# Autodesk Inventor assembly: Front support bearing and stopper
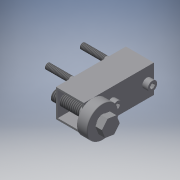
[picture p0: Inventor's stored thumbnail of the model, 180x180]
Saved by Autodesk Inventor 2018 (Build 220112000, 112)
## iProperties
Created: 2019-03-22
Part Number: Front support bearing and stopper
Document SubType Name: Assembly
Designer: s-4008082
Author: s-4008082
## Documents named in this file (6)
- \\studenthome\students\S-4008082\robotics\Front support bearing and stopper.iam
- \\studenthome\students\S-4008082\robotics\Front support bearing and stopper.ipt
- \\studenthome\students\S-4008082\robotics\10 l 20 2 1 l 2 bolt.ipt
- \\studenthome\students\S-4008082\robotics\1614zz bearing.ipt
- \\studenthome\students\S-4008082\robotics\3 l 8 Bolt.ipt
- \\studenthome\students\S-4008082\robotics\.05 spacer.ipt
## Components (7 placed, 5 different names)
1. Front support bearing and stopper:1 — Mate:4, Mate:5, Mate:6, Mate:7, Mate:9
2. 10 l 20 2 1 l 2 bolt:1 — Mate:4, Mate:7
3. 1614zz bearing:1 — Mate:8, Mate:12, Mate:14
4. 3 l 8 Bolt:1 — Mate:8, Mate:10, Mate:11, Mate:13
5. 10 l 20 2 1 l 2 bolt:2 — Mate:5, Mate:6
6. .05 spacer:1 — Mate:9, Mate:10, Mate:14
7. .05 spacer:2 — Mate:11, Mate:12, Mate:13
## Relationships (11: Mate 11)
- Mate:4: Front support bearing and stopper:1 ↔ 10 l 20 2 1 l 2 bolt:1
- Mate:5: Front support bearing and stopper:1 ↔ 10 l 20 2 1 l 2 bolt:2
- Mate:6: Front support bearing and stopper:1 ↔ 10 l 20 2 1 l 2 bolt:2
- Mate:7: Front support bearing and stopper:1 ↔ 10 l 20 2 1 l 2 bolt:1
- Mate:8: 1614zz bearing:1 ↔ 3 l 8 Bolt:1
- Mate:9: Front support bearing and stopper:1 ↔ .05 spacer:1
- Mate:10: 3 l 8 Bolt:1 ↔ .05 spacer:1
- Mate:11: 3 l 8 Bolt:1 ↔ .05 spacer:2
- Mate:12: 1614zz bearing:1 ↔ .05 spacer:2
- Mate:13: 3 l 8 Bolt:1 ↔ .05 spacer:2
- Mate:14: 1614zz bearing:1 ↔ .05 spacer:1
